# Autodesk Inventor assembly: polivalka
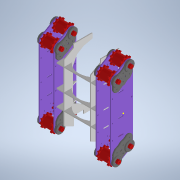
[picture p0: Inventor's stored thumbnail of the model, 180x180]
Saved by Autodesk Inventor 2022 (Build 260153000, 153)
## iProperties
Created: 2022-10-22
Part Number: polivalka
Document SubType Name: Assembly
Designer: КозьминАндрей
Author: КозьминАндрей
## Documents named in this file (4)
- D:\Проэкты Autodesk Inventor\polivalka\Sborki\polivalka.iam
- D:\Проэкты Autodesk Inventor\polivalka\Sborki\ramaGusenitsi.iam
- D:\Проэкты Autodesk Inventor\polivalka\myDno.ipt
- D:\Проэкты Autodesk Inventor\polivalka\balkaRami.ipt
## Components (7 placed, 3 different names)
1. ramaGusenitsi:1 [sub-assembly] — Совмещение:2, Совмещение:3, Совмещение:4, Совмещение:7, Совмещение:8, Совмещение:9, Совмещение:10, Совмещение:11, Совмещение:12
2. ramaGusenitsi:2 [sub-assembly] — Совмещение:1, Совмещение:5, Совмещение:6
3. myDno:1 — Совмещение:1, Совмещение:2, Совмещение:3, Совмещение:4, Совмещение:5, Совмещение:6, Совмещение:13, Совмещение:14, Совмещение:15, Совмещение:16
4. myDno:2 — Совмещение:10, Совмещение:11, Совмещение:12
5. myDno:3 — Совмещение:7, Совмещение:8, Совмещение:9
6. balkaRami:1 — Совмещение:13, Совмещение:14
7. balkaRami:2 — Совмещение:15, Совмещение:16
## Relationships (16: Mate 16)
- Совмещение:1 [Mate]: ramaGusenitsi:2 ↔ myDno:1
- Совмещение:2 [Mate]: ramaGusenitsi:1 ↔ myDno:1
- Совмещение:3 [Mate]: ramaGusenitsi:1 ↔ myDno:1
- Совмещение:4 [Mate]: ramaGusenitsi:1 ↔ myDno:1
- Совмещение:5 [Mate]: ramaGusenitsi:2 ↔ myDno:1
- Совмещение:6 [Mate]: ramaGusenitsi:2 ↔ myDno:1
- Совмещение:7 [Mate]: ramaGusenitsi:1 ↔ myDno:3
- Совмещение:8 [Mate]: ramaGusenitsi:1 ↔ myDno:3
- Совмещение:9 [Mate]: ramaGusenitsi:1 ↔ myDno:3
- Совмещение:10 [Mate]: ramaGusenitsi:1 ↔ myDno:2
- Совмещение:11 [Mate]: ramaGusenitsi:1 ↔ myDno:2
- Совмещение:12 [Mate]: ramaGusenitsi:1 ↔ myDno:2
- Совмещение:13 [Mate]: myDno:1 ↔ balkaRami:1
- Совмещение:14 [Mate]: myDno:1 ↔ balkaRami:1
- Совмещение:15 [Mate]: myDno:1 ↔ balkaRami:2
- Совмещение:16 [Mate]: myDno:1 ↔ balkaRami:2
